# Autodesk Inventor assembly: ReelAssembly_SBail
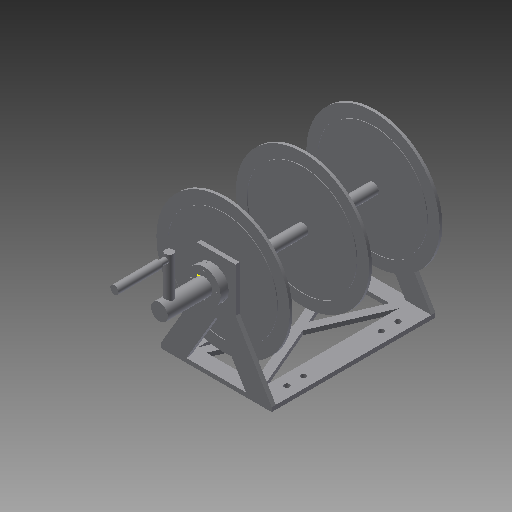
[picture p0: Inventor's stored thumbnail of the model, 512x512]
Saved by Autodesk Inventor 2019 (Build 230136000, 136)
## iProperties
Created: 2019-04-17
Part Number: ReelAssembly_SBail
Document SubType Name: Assembly
Designer: samson.bailor
Author: samson.bailor
## Documents named in this file (11)
- S:\Modern Technology Academy\Bogdziewicz\Student Drop Box\1-Collaboration\47-EDD-2019\Trotline\trotline-reel\src\inventor\ReelAssembly_SBail.iam
- S:\Modern Technology Academy\Bogdziewicz\Student Drop Box\1-Collaboration\47-EDD-2019\Trotline\trotline-reel\src\inventor\Axle_SBail.ipt
- S:\Modern Technology Academy\Bogdziewicz\Student Drop Box\1-Collaboration\47-EDD-2019\Trotline\trotline-reel\src\inventor\Plate.ipt
- S:\Modern Technology Academy\Bogdziewicz\Student Drop Box\1-Collaboration\47-EDD-2019\Trotline\trotline-reel\src\inventor\PlateCenter.ipt
- S:\Modern Technology Academy\Bogdziewicz\Student Drop Box\1-Collaboration\47-EDD-2019\Trotline\trotline-reel\src\inventor\Square Support.ipt
- S:\Modern Technology Academy\Bogdziewicz\Student Drop Box\1-Collaboration\47-EDD-2019\Trotline\trotline-reel\src\inventor\CrankHandle_SBail.ipt
- S:\Modern Technology Academy\Bogdziewicz\Student Drop Box\1-Collaboration\47-EDD-2019\Trotline\trotline-reel\src\inventor\CrankP1_SBail.ipt
- S:\Modern Technology Academy\Bogdziewicz\Student Drop Box\1-Collaboration\47-EDD-2019\Trotline\trotline-reel\src\inventor\CrankP2_SBail.ipt
- S:\Modern Technology Academy\Bogdziewicz\Student Drop Box\1-Collaboration\47-EDD-2019\Trotline\trotline-reel\src\inventor\Ball_Bearing_KFuchs.ipt
- S:\Modern Technology Academy\Bogdziewicz\Student Drop Box\1-Collaboration\47-EDD-2019\Trotline\trotline-reel\src\inventor\CrankAttachment_SBail.ipt
- S:\Modern Technology Academy\Bogdziewicz\Student Drop Box\1-Collaboration\47-EDD-2019\Trotline\trotline-reel\src\inventor\Bolt_SBail.ipt
## Components (15 placed, 10 different names)
1. Axle_SBail:1 — Mate:3, Insert:1, Insert:2, Insert:3, Insert:8
2. PlateCenter:1 — Mate:3
3. Plate:3 — Insert:1
4. Plate:4 — Insert:2
5. Square Support:1 — Insert:3, Insert:6, Insert:7
6. CrankHandle_SBail:1 — Mate:4
7. CrankP2_SBail:1 — Mate:4, Insert:10
8. Ball_Bearing_KFuchs:1 — Insert:7
9. Ball_Bearing_KFuchs:2 — Insert:6
10. CrankAttachment_SBail:1 — Insert:8, Insert:9
11. CrankP1_SBail:1 — Insert:9, Insert:10, Insert:11, Insert:12, Insert:13, Insert:14
12. Bolt_SBail:1 — Insert:12
13. Bolt_SBail:2 — Insert:13
14. Bolt_SBail:3 — Insert:11
15. Bolt_SBail:4 — Insert:14
## Relationships (14: Insert 12, Mate 2)
- Mate:3: Axle_SBail:1 ↔ PlateCenter:1
- Insert:1: Axle_SBail:1 ↔ Plate:3
- Insert:2: Axle_SBail:1 ↔ Plate:4
- Insert:3: Axle_SBail:1 ↔ Square Support:1
- Mate:4: CrankHandle_SBail:1 ↔ CrankP2_SBail:1
- Insert:6: Square Support:1 ↔ Ball_Bearing_KFuchs:2
- Insert:7: Square Support:1 ↔ Ball_Bearing_KFuchs:1
- Insert:8: Axle_SBail:1 ↔ CrankAttachment_SBail:1
- Insert:9: CrankAttachment_SBail:1 ↔ CrankP1_SBail:1
- Insert:10: CrankP2_SBail:1 ↔ CrankP1_SBail:1
- Insert:11: CrankP1_SBail:1 ↔ Bolt_SBail:3
- Insert:12: CrankP1_SBail:1 ↔ Bolt_SBail:1
- Insert:13: CrankP1_SBail:1 ↔ Bolt_SBail:2
- Insert:14: CrankP1_SBail:1 ↔ Bolt_SBail:4
